# Autodesk Inventor assembly: config - graphic card asm
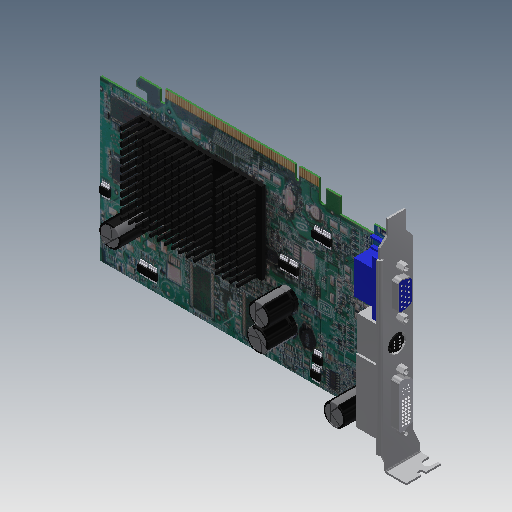
[picture p0: Inventor's stored thumbnail of the model, 512x512]
Saved by Autodesk Inventor 2020 (Build 240152000, 152)
## iProperties
Company: Autodesk Asia Pte. Ltd.
Created: 2005-12-11
Part Number: config - graphic card asm
Document SubType Name: Assembly
Designer: Simon.Ng@autodesk.com
Stock Number: NA
Description: Graphic Interface
Mass: 53.2227 g
Surface Area: 677.743 cm^2
Volume: 53.2227 cm^3
Density: 1 g/cm^3
Title: Purchased Part
Author: Simon.Ng@autodesk.com
Revision Number: A
## Documents named in this file (7)
- C:\Users\hallc\Desktop\Process Equipment\Workspace\Supplier Content\Electrical Design\Graphics Card\Graphics Card.iam
- C:\Users\hallc\Desktop\Process Equipment\Workspace\Supplier Content\Electrical Design\Graphics Card\Graphic Card PCB.ipt
- C:\Users\hallc\Desktop\Process Equipment\Workspace\Supplier Content\Electrical Design\Graphics Card\Graphic Card Heat Sink.ipt
- C:\Users\hallc\Desktop\Process Equipment\Workspace\Supplier Content\Electrical Design\Motherboard\Chip 5 x 3.ipt
- C:\Users\hallc\Desktop\Process Equipment\Workspace\Supplier Content\Electrical Design\Motherboard\Capacitor 3500 UF.ipt
- C:\Users\hallc\Desktop\Process Equipment\Workspace\Supplier Content\Electrical Design\Motherboard\Chip 22 x 11.ipt
- C:\Users\hallc\Desktop\Process Equipment\Workspace\Supplier Content\Electrical Design\Graphics Card\Graphic Card Sheetmetal.ipt
## Components (18 placed, 6 different names)
1. Graphic Card PCB:1 — Mate:1, Mate:2, Mate:3, Mate:4, Mate:5, Mate:6, Mate:7, Mate:8, Mate:9, Mate:10, Mate:11, Mate:12, Mate:13, Mate:14, Mate:15, Mate:16, Flush:2, Mate:18, Mate:19
2. Capacitor 3500 UF:1 — Mate:1
3. Capacitor 3500 UF:2 — Mate:2
4. Capacitor 3500 UF:3 — Mate:3
5. Graphic Card Heat Sink:1 — Mate:4
6. Capacitor 3500 UF:4 — Mate:5
7. Chip 5 x 3:1 — Mate:8
8. Chip 5 x 3:2 — Mate:7
9. Chip 5 x 3:3 — Mate:6
10. Chip 5 x 3:4 — Mate:9
11. Chip 5 x 3:5 — Mate:10
12. Chip 22 x 11:1 — Mate:11
13. Chip 22 x 11:2 — Mate:12
14. Chip 5 x 3:6 — Mate:13
15. Chip 5 x 3:7 — Mate:14
16. Chip 5 x 3:8 — Mate:15, Flush:1
17. Chip 5 x 3:9 — Mate:16, Flush:1
18. Graphic Card Sheetmetal:1 — Flush:2, Mate:18, Mate:19
## Relationships (20: Mate 18, Flush 2)
- Mate:1: Graphic Card PCB:1 ↔ Capacitor 3500 UF:1
- Mate:2: Graphic Card PCB:1 ↔ Capacitor 3500 UF:2
- Mate:3: Graphic Card PCB:1 ↔ Capacitor 3500 UF:3
- Mate:4: Graphic Card PCB:1 ↔ Graphic Card Heat Sink:1
- Mate:5: Graphic Card PCB:1 ↔ Capacitor 3500 UF:4
- Mate:6: Graphic Card PCB:1 ↔ Chip 5 x 3:3
- Mate:7: Graphic Card PCB:1 ↔ Chip 5 x 3:2
- Mate:8: Graphic Card PCB:1 ↔ Chip 5 x 3:1
- Mate:9: Graphic Card PCB:1 ↔ Chip 5 x 3:4
- Mate:10: Graphic Card PCB:1 ↔ Chip 5 x 3:5
- Mate:11: Graphic Card PCB:1 ↔ Chip 22 x 11:1
- Mate:12: Graphic Card PCB:1 ↔ Chip 22 x 11:2
- Mate:13: Graphic Card PCB:1 ↔ Chip 5 x 3:6
- Mate:14: Graphic Card PCB:1 ↔ Chip 5 x 3:7
- Mate:15: Graphic Card PCB:1 ↔ Chip 5 x 3:8
- Mate:16: Graphic Card PCB:1 ↔ Chip 5 x 3:9
- Flush:1: Chip 5 x 3:8 ↔ Chip 5 x 3:9
- Flush:2 (4 mm): Graphic Card PCB:1 ↔ Graphic Card Sheetmetal:1
- Mate:18 (1 mm): Graphic Card PCB:1 ↔ Graphic Card Sheetmetal:1
- Mate:19: Graphic Card PCB:1 ↔ Graphic Card Sheetmetal:1
